# Autodesk Inventor assembly: Assembly3
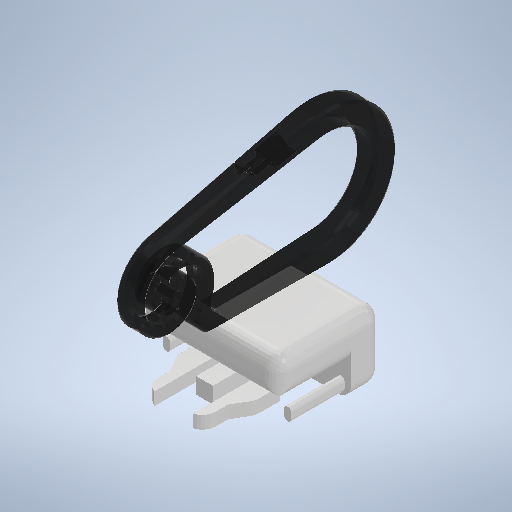
[picture p0: Inventor's stored thumbnail of the model, 512x512]
Saved by Autodesk Inventor 2025 (Build 290162010, 162A)
## iProperties
Created: 2026-05-19
Part Number: Assembly3
Document SubType Name: Assembly
Designer: 925699
Author: 925699
## Documents named in this file (3)
- C:\Users\925699\Documents\Inventor\Spirabiner\Assembly3.iam
- C:\Users\925699\Documents\Inventor\Spirabiner\Part6.ipt
- C:\Users\925699\Documents\Inventor\Spirabiner\Part1.ipt
## Components (2 placed, 2 different names)
1. Part6:1 — Rotational:1
2. Part1:1 — Rotational:1
## Relationships (1: RevoluteJoint 1)
- Rotational:1 [RevoluteJoint]: Part6:1 ↔ Part1:1
